# Autodesk Inventor assembly: 装配-载板集合
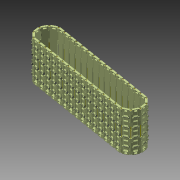
[picture p0: Inventor's stored thumbnail of the model, 180x180]
Saved by Autodesk Inventor 2015 (Build 190159000, 159)
## iProperties
Created: 2017-05-23
Part Number: 装配-载板集合
Document SubType Name: Assembly
Designer: Administrator
Author: Administrator
## Documents named in this file (4)
- C:\Users\Administrator\Desktop\毕设改\装配-载板集合.iam
- C:\Users\Administrator\Desktop\毕设改\装配-载板.iam
- C:\Users\Administrator\Desktop\毕设改\夹具固定销.ipt
- C:\Users\Administrator\Desktop\毕设改\夹具固定销螺丝.ipt
## Components (798 placed, 3 different names)
1. 装配-载板:2 [sub-assembly] — 插入:1, 角度:1, 插入:2, 角度:2, 插入:43, 表面齐平:3
2. 装配-载板:3 [sub-assembly] — 插入:2, 角度:2, 插入:3, 角度:3, 插入:38, 表面齐平:2
3. 装配-载板:4 [sub-assembly] — 插入:3, 插入:4, 角度:3, 角度:4, 插入:36, 插入:37
4. 装配-载板:5 [sub-assembly] — 插入:4, 插入:5, 角度:4, 插入:35, 表面齐平:1
5. 装配-载板:7 [sub-assembly] — 插入:6, 角度:5, 插入:7, 角度:6, 插入:62, 配合:1
6. 装配-载板:8 [sub-assembly] — 插入:6, 角度:5, 插入:9, 插入:60, 插入:61
7. 装配-载板:37 [sub-assembly] — 插入:7, 角度:6, 插入:8, 角度:7, 插入:63, 表面齐平:4
8. 装配-载板:38 [sub-assembly] — 插入:8, 角度:7, 插入:10, 插入:64, 表面齐平:5
9. 装配-载板:1 [sub-assembly] — 插入:1, 角度:1
10. 装配-载板:9 [sub-assembly]
11. 装配-载板:10 [sub-assembly]
12. 装配-载板:11 [sub-assembly]
13. 装配-载板:12 [sub-assembly]
14. 装配-载板:13 [sub-assembly]
15. 装配-载板:14 [sub-assembly]
16. 装配-载板:15 [sub-assembly]
17. 装配-载板:16 [sub-assembly]
18. 装配-载板:17 [sub-assembly]
19. 装配-载板:18 [sub-assembly]
20. 装配-载板:19 [sub-assembly]
21. 装配-载板:20 [sub-assembly]
22. 装配-载板:21 [sub-assembly]
23. 装配-载板:22 [sub-assembly] — 插入:10, 插入:21, 插入:22
24. 装配-载板:6 [sub-assembly] — 插入:5, 插入:11, 插入:12
25. 装配-载板:23 [sub-assembly]
26. 装配-载板:24 [sub-assembly]
27. 装配-载板:25 [sub-assembly]
28. 装配-载板:26 [sub-assembly]
29. 装配-载板:27 [sub-assembly]
30. 装配-载板:28 [sub-assembly]
31. 装配-载板:29 [sub-assembly]
32. 装配-载板:30 [sub-assembly]
33. 装配-载板:31 [sub-assembly]
34. 装配-载板:32 [sub-assembly]
35. 装配-载板:33 [sub-assembly]
36. 装配-载板:34 [sub-assembly]
37. 装配-载板:35 [sub-assembly]
38. 装配-载板:36 [sub-assembly] — 插入:9
39. 夹具固定销:130 — 插入:60, 插入:61
40. 夹具固定销螺丝:502
41. 夹具固定销螺丝:503
42. 夹具固定销螺丝:505
43. 夹具固定销螺丝:504
44. 夹具固定销:133 — 插入:62, 配合:1
45. 夹具固定销螺丝:515
46. 夹具固定销螺丝:514
47. 夹具固定销螺丝:517
48. 夹具固定销螺丝:516
49. 夹具固定销:132 — 插入:64, 表面齐平:5
50. 夹具固定销螺丝:510
51. 夹具固定销螺丝:511
52. 夹具固定销螺丝:513
53. 夹具固定销螺丝:512
54. 夹具固定销:131 — 插入:63, 表面齐平:4
55. 夹具固定销螺丝:506
56. 夹具固定销螺丝:507
57. 夹具固定销螺丝:509
58. 夹具固定销螺丝:508
59. 夹具固定销:128 — 插入:38, 表面齐平:2
60. 夹具固定销螺丝:494
61. 夹具固定销螺丝:495
62. 夹具固定销螺丝:496
63. 夹具固定销螺丝:497
64. 夹具固定销:129 — 插入:43, 表面齐平:3
65. 夹具固定销螺丝:498
66. 夹具固定销螺丝:499
67. 夹具固定销螺丝:501
68. 夹具固定销螺丝:500
69. 夹具固定销:2 — 插入:23, 插入:24, 插入:25, 插入:26, 插入:35, 表面齐平:1
70. 夹具固定销螺丝:2 — 插入:23
71. 夹具固定销螺丝:487 — 插入:26
72. 夹具固定销螺丝:489 — 插入:25
73. 夹具固定销螺丝:488 — 插入:24
74. 夹具固定销:127 — 插入:36, 插入:37
75. 夹具固定销螺丝:490
76. 夹具固定销螺丝:491
77. 夹具固定销螺丝:493
78. 夹具固定销螺丝:492
79. 夹具固定销:134
80. 夹具固定销螺丝:518
81. 夹具固定销螺丝:519
82. 夹具固定销螺丝:520
83. 夹具固定销螺丝:521
84. 夹具固定销:135
85. 夹具固定销螺丝:522
86. 夹具固定销螺丝:523
87. 夹具固定销螺丝:524
88. 夹具固定销螺丝:525
89. 夹具固定销:136
90. 夹具固定销螺丝:526
91. 夹具固定销螺丝:527
92. 夹具固定销螺丝:528
93. 夹具固定销螺丝:529
94. 夹具固定销:137
95. 夹具固定销螺丝:530
96. 夹具固定销螺丝:531
97. 夹具固定销螺丝:532
98. 夹具固定销螺丝:533
99. 夹具固定销:138
100. 夹具固定销螺丝:534
101. 夹具固定销螺丝:535
102. 夹具固定销螺丝:536
103. 夹具固定销螺丝:537
104. 夹具固定销:139
105. 夹具固定销螺丝:538
106. 夹具固定销螺丝:539
107. 夹具固定销螺丝:540
108. 夹具固定销螺丝:541
109. 夹具固定销:140
110. 夹具固定销螺丝:542
111. 夹具固定销螺丝:543
112. 夹具固定销螺丝:544
113. 夹具固定销螺丝:545
114. 夹具固定销:141
115. 夹具固定销螺丝:546
116. 夹具固定销螺丝:547
117. 夹具固定销螺丝:548
118. 夹具固定销螺丝:549
119. 夹具固定销:142
120. 夹具固定销螺丝:550
121. 夹具固定销螺丝:551
122. 夹具固定销螺丝:552
123. 夹具固定销螺丝:553
124. 夹具固定销:143
125. 夹具固定销螺丝:554
126. 夹具固定销螺丝:555
127. 夹具固定销螺丝:556
128. 夹具固定销螺丝:557
129. 夹具固定销:144
130. 夹具固定销螺丝:558
131. 夹具固定销螺丝:559
132. 夹具固定销螺丝:560
133. 夹具固定销螺丝:561
134. 夹具固定销:145
135. 夹具固定销螺丝:562
136. 夹具固定销螺丝:563
137. 夹具固定销螺丝:564
138. 夹具固定销螺丝:565
139. 夹具固定销:146
140. 夹具固定销螺丝:566
141. 夹具固定销螺丝:567
142. 夹具固定销螺丝:568
143. 夹具固定销螺丝:569
144. 夹具固定销:147
145. 夹具固定销螺丝:570
146. 夹具固定销螺丝:571
147. 夹具固定销螺丝:572
148. 夹具固定销螺丝:573
149. 夹具固定销:148
150. 夹具固定销螺丝:574
151. 夹具固定销螺丝:575
152. 夹具固定销螺丝:576
153. 夹具固定销螺丝:577
154. 夹具固定销:149
155. 夹具固定销螺丝:578
156. 夹具固定销螺丝:579
157. 夹具固定销螺丝:580
158. 夹具固定销螺丝:581
159. 夹具固定销:150
160. 夹具固定销螺丝:582
161. 夹具固定销螺丝:583
162. 夹具固定销螺丝:584
163. 夹具固定销螺丝:585
164. 夹具固定销:151
165. 夹具固定销螺丝:586
166. 夹具固定销螺丝:587
167. 夹具固定销螺丝:588
168. 夹具固定销螺丝:589
169. 夹具固定销:152
170. 夹具固定销螺丝:590
171. 夹具固定销螺丝:591
172. 夹具固定销螺丝:592
173. 夹具固定销螺丝:593
174. 夹具固定销:153
175. 夹具固定销螺丝:594
176. 夹具固定销螺丝:595
177. 夹具固定销螺丝:596
178. 夹具固定销螺丝:597
179. 夹具固定销:154
180. 夹具固定销螺丝:598
181. 夹具固定销螺丝:599
182. 夹具固定销螺丝:600
183. 夹具固定销螺丝:601
184. 夹具固定销:155
185. 夹具固定销螺丝:602
186. 夹具固定销螺丝:603
187. 夹具固定销螺丝:604
188. 夹具固定销螺丝:605
189. 夹具固定销:156
190. 夹具固定销螺丝:606
191. 夹具固定销螺丝:607
192. 夹具固定销螺丝:608
193. 夹具固定销螺丝:609
194. 夹具固定销:157
195. 夹具固定销螺丝:610
196. 夹具固定销螺丝:611
197. 夹具固定销螺丝:612
198. 夹具固定销螺丝:613
199. 夹具固定销:5 — 插入:11, 插入:12, 插入:13, 插入:14, 插入:15, 插入:16
200. 夹具固定销螺丝:5 — 插入:13
201. 夹具固定销螺丝:10 — 插入:15
202. 夹具固定销螺丝:11 — 插入:16
203. 夹具固定销螺丝:9 — 插入:14
204. 夹具固定销:9
205. 夹具固定销螺丝:12
206. 夹具固定销螺丝:13
207. 夹具固定销螺丝:14
208. 夹具固定销螺丝:15
209. 夹具固定销:10
210. 夹具固定销螺丝:16
211. 夹具固定销螺丝:17
212. 夹具固定销螺丝:18
213. 夹具固定销螺丝:19
214. 夹具固定销:11
215. 夹具固定销螺丝:20
216. 夹具固定销螺丝:21
217. 夹具固定销螺丝:22
218. 夹具固定销螺丝:23
219. 夹具固定销:12
220. 夹具固定销螺丝:24
221. 夹具固定销螺丝:25
222. 夹具固定销螺丝:26
223. 夹具固定销螺丝:27
224. 夹具固定销:13
225. 夹具固定销螺丝:28
226. 夹具固定销螺丝:29
227. 夹具固定销螺丝:30
228. 夹具固定销螺丝:31
229. 夹具固定销:14
230. 夹具固定销螺丝:32
231. 夹具固定销螺丝:33
232. 夹具固定销螺丝:34
233. 夹具固定销螺丝:35
234. 夹具固定销:15
235. 夹具固定销螺丝:36
236. 夹具固定销螺丝:37
237. 夹具固定销螺丝:38
238. 夹具固定销螺丝:39
239. 夹具固定销:16
240. 夹具固定销螺丝:40
241. 夹具固定销螺丝:41
242. 夹具固定销螺丝:42
243. 夹具固定销螺丝:43
244. 夹具固定销:17
245. 夹具固定销螺丝:44
246. 夹具固定销螺丝:45
247. 夹具固定销螺丝:46
248. 夹具固定销螺丝:47
249. 夹具固定销:18
250. 夹具固定销螺丝:48
251. 夹具固定销螺丝:49
252. 夹具固定销螺丝:50
253. 夹具固定销螺丝:51
254. 夹具固定销:19
255. 夹具固定销螺丝:52
256. 夹具固定销螺丝:53
257. 夹具固定销螺丝:54
258. 夹具固定销螺丝:55
259. 夹具固定销:20
260. 夹具固定销螺丝:56
261. 夹具固定销螺丝:57
262. 夹具固定销螺丝:58
263. 夹具固定销螺丝:59
264. 夹具固定销:21
265. 夹具固定销螺丝:60
266. 夹具固定销螺丝:61
267. 夹具固定销螺丝:62
268. 夹具固定销螺丝:63
269. 夹具固定销:22
270. 夹具固定销螺丝:64
271. 夹具固定销螺丝:65
272. 夹具固定销螺丝:66
273. 夹具固定销螺丝:67
274. 夹具固定销:23
275. 夹具固定销螺丝:68
276. 夹具固定销螺丝:69
277. 夹具固定销螺丝:70
278. 夹具固定销螺丝:71
279. 夹具固定销:24
280. 夹具固定销螺丝:72
281. 夹具固定销螺丝:73
282. 夹具固定销螺丝:74
283. 夹具固定销螺丝:75
284. 夹具固定销:25
285. 夹具固定销螺丝:76
286. 夹具固定销螺丝:77
287. 夹具固定销螺丝:78
288. 夹具固定销螺丝:79
289. 夹具固定销:26
290. 夹具固定销螺丝:80
291. 夹具固定销螺丝:81
292. 夹具固定销螺丝:82
293. 夹具固定销螺丝:83
294. 夹具固定销:27
295. 夹具固定销螺丝:84
296. 夹具固定销螺丝:85
297. 夹具固定销螺丝:86
298. 夹具固定销螺丝:87
299. 夹具固定销:28
300. 夹具固定销螺丝:88
301. 夹具固定销螺丝:89
302. 夹具固定销螺丝:90
303. 夹具固定销螺丝:91
304. 夹具固定销:29
305. 夹具固定销螺丝:92
306. 夹具固定销螺丝:93
307. 夹具固定销螺丝:94
308. 夹具固定销螺丝:95
309. 夹具固定销:30
310. 夹具固定销螺丝:96
311. 夹具固定销螺丝:97
312. 夹具固定销螺丝:98
313. 夹具固定销螺丝:99
314. 夹具固定销:31
315. 夹具固定销螺丝:100
316. 夹具固定销螺丝:101
317. 夹具固定销螺丝:102
318. 夹具固定销螺丝:103
319. 夹具固定销:32
320. 夹具固定销螺丝:104
321. 夹具固定销螺丝:105
322. 夹具固定销螺丝:106
323. 夹具固定销螺丝:107
324. 夹具固定销:33
325. 夹具固定销螺丝:108
326. 夹具固定销螺丝:109
327. 夹具固定销螺丝:110
328. 夹具固定销螺丝:111
329. 夹具固定销:34
330. 夹具固定销螺丝:112
331. 夹具固定销螺丝:113
332. 夹具固定销螺丝:114
333. 夹具固定销螺丝:115
334. 夹具固定销:35
335. 夹具固定销螺丝:116
336. 夹具固定销螺丝:117
337. 夹具固定销螺丝:118
338. 夹具固定销螺丝:119
339. 夹具固定销:36
340. 夹具固定销螺丝:120
341. 夹具固定销螺丝:121
342. 夹具固定销螺丝:122
343. 夹具固定销螺丝:123
344. 夹具固定销:37
345. 夹具固定销螺丝:124
346. 夹具固定销螺丝:125
347. 夹具固定销螺丝:126
348. 夹具固定销螺丝:127
349. 夹具固定销:38
350. 夹具固定销螺丝:128
351. 夹具固定销螺丝:129
352. 夹具固定销螺丝:130
353. 夹具固定销螺丝:131
354. 夹具固定销:39
355. 夹具固定销螺丝:132
356. 夹具固定销螺丝:133
357. 夹具固定销螺丝:134
358. 夹具固定销螺丝:135
359. 夹具固定销:40
360. 夹具固定销螺丝:136
361. 夹具固定销螺丝:137
362. 夹具固定销螺丝:138
363. 夹具固定销螺丝:139
364. 夹具固定销:41
365. 夹具固定销螺丝:140
366. 夹具固定销螺丝:141
367. 夹具固定销螺丝:142
368. 夹具固定销螺丝:143
369. 夹具固定销:42
370. 夹具固定销螺丝:144
371. 夹具固定销螺丝:145
372. 夹具固定销螺丝:146
373. 夹具固定销螺丝:147
374. 夹具固定销:43
375. 夹具固定销螺丝:148
376. 夹具固定销螺丝:149
377. 夹具固定销螺丝:150
378. 夹具固定销螺丝:151
379. 夹具固定销:44
380. 夹具固定销螺丝:152
381. 夹具固定销螺丝:153
382. 夹具固定销螺丝:154
383. 夹具固定销螺丝:155
384. 夹具固定销:45
385. 夹具固定销螺丝:156
386. 夹具固定销螺丝:157
387. 夹具固定销螺丝:158
388. 夹具固定销螺丝:159
389. 夹具固定销:46
390. 夹具固定销螺丝:160
391. 夹具固定销螺丝:161
392. 夹具固定销螺丝:162
393. 夹具固定销螺丝:163
394. 夹具固定销:47
395. 夹具固定销螺丝:164
396. 夹具固定销螺丝:165
397. 夹具固定销螺丝:166
398. 夹具固定销螺丝:167
399. 夹具固定销:48
400. 夹具固定销螺丝:168
401. 夹具固定销螺丝:169
402. 夹具固定销螺丝:170
403. 夹具固定销螺丝:171
404. 夹具固定销:49
405. 夹具固定销螺丝:172
406. 夹具固定销螺丝:173
407. 夹具固定销螺丝:174
408. 夹具固定销螺丝:175
409. 夹具固定销:50
410. 夹具固定销螺丝:176
411. 夹具固定销螺丝:177
412. 夹具固定销螺丝:178
413. 夹具固定销螺丝:179
414. 夹具固定销:51
415. 夹具固定销螺丝:180
416. 夹具固定销螺丝:181
417. 夹具固定销螺丝:182
418. 夹具固定销螺丝:183
419. 夹具固定销:52
420. 夹具固定销螺丝:184
421. 夹具固定销螺丝:185
422. 夹具固定销螺丝:186
423. 夹具固定销螺丝:187
424. 夹具固定销:53
425. 夹具固定销螺丝:188
426. 夹具固定销螺丝:189
427. 夹具固定销螺丝:190
428. 夹具固定销螺丝:191
429. 夹具固定销:54
430. 夹具固定销螺丝:192
431. 夹具固定销螺丝:193
432. 夹具固定销螺丝:194
433. 夹具固定销螺丝:195
434. 夹具固定销:55
435. 夹具固定销螺丝:196
436. 夹具固定销螺丝:197
437. 夹具固定销螺丝:198
438. 夹具固定销螺丝:199
439. 夹具固定销:56
440. 夹具固定销螺丝:200
441. 夹具固定销螺丝:201
442. 夹具固定销螺丝:202
443. 夹具固定销螺丝:203
444. 夹具固定销:57
445. 夹具固定销螺丝:204
446. 夹具固定销螺丝:205
447. 夹具固定销螺丝:206
448. 夹具固定销螺丝:207
449. 夹具固定销:58
450. 夹具固定销螺丝:208
451. 夹具固定销螺丝:209
452. 夹具固定销螺丝:210
453. 夹具固定销螺丝:211
454. 夹具固定销:59
455. 夹具固定销螺丝:212
456. 夹具固定销螺丝:213
457. 夹具固定销螺丝:214
458. 夹具固定销螺丝:215
459. 夹具固定销:60
460. 夹具固定销螺丝:216
461. 夹具固定销螺丝:217
462. 夹具固定销螺丝:218
463. 夹具固定销螺丝:219
464. 夹具固定销:61
465. 夹具固定销螺丝:220
466. 夹具固定销螺丝:221
467. 夹具固定销螺丝:222
468. 夹具固定销螺丝:223
469. 夹具固定销:62
470. 夹具固定销螺丝:224
471. 夹具固定销螺丝:225
472. 夹具固定销螺丝:226
473. 夹具固定销螺丝:227
474. 夹具固定销:63
475. 夹具固定销螺丝:228
476. 夹具固定销螺丝:229
477. 夹具固定销螺丝:230
478. 夹具固定销螺丝:231
479. 夹具固定销:64
480. 夹具固定销螺丝:232
481. 夹具固定销螺丝:233
482. 夹具固定销螺丝:234
483. 夹具固定销螺丝:235
484. 夹具固定销:65
485. 夹具固定销螺丝:236
486. 夹具固定销螺丝:237
487. 夹具固定销螺丝:238
488. 夹具固定销螺丝:239
489. 夹具固定销:66
490. 夹具固定销螺丝:240
491. 夹具固定销螺丝:241
492. 夹具固定销螺丝:242
493. 夹具固定销螺丝:243
494. 夹具固定销:67
495. 夹具固定销螺丝:244
496. 夹具固定销螺丝:245
497. 夹具固定销螺丝:246
498. 夹具固定销螺丝:247
499. 夹具固定销:1 — 插入:17, 插入:18, 插入:19, 插入:20, 插入:21, 插入:22
500. 夹具固定销螺丝:249 — 插入:18
501. 夹具固定销螺丝:1 — 插入:17
502. 夹具固定销螺丝:250 — 插入:20
503. 夹具固定销螺丝:248 — 插入:19
504. 夹具固定销:68
505. 夹具固定销螺丝:251
506. 夹具固定销螺丝:252
507. 夹具固定销螺丝:253
508. 夹具固定销螺丝:254
509. 夹具固定销:69
510. 夹具固定销螺丝:255
511. 夹具固定销螺丝:256
512. 夹具固定销螺丝:257
513. 夹具固定销螺丝:258
514. 夹具固定销:70
515. 夹具固定销螺丝:259
516. 夹具固定销螺丝:260
517. 夹具固定销螺丝:261
518. 夹具固定销螺丝:262
519. 夹具固定销:71
520. 夹具固定销螺丝:263
521. 夹具固定销螺丝:264
522. 夹具固定销螺丝:265
523. 夹具固定销螺丝:266
524. 夹具固定销:72
525. 夹具固定销螺丝:267
526. 夹具固定销螺丝:268
527. 夹具固定销螺丝:269
528. 夹具固定销螺丝:270
529. 夹具固定销:73
530. 夹具固定销螺丝:271
531. 夹具固定销螺丝:272
532. 夹具固定销螺丝:273
533. 夹具固定销螺丝:274
534. 夹具固定销:74
535. 夹具固定销螺丝:275
536. 夹具固定销螺丝:276
537. 夹具固定销螺丝:277
538. 夹具固定销螺丝:278
539. 夹具固定销:75
540. 夹具固定销螺丝:279
541. 夹具固定销螺丝:280
542. 夹具固定销螺丝:281
543. 夹具固定销螺丝:282
544. 夹具固定销:76
545. 夹具固定销螺丝:283
546. 夹具固定销螺丝:284
547. 夹具固定销螺丝:285
548. 夹具固定销螺丝:286
549. 夹具固定销:77
550. 夹具固定销螺丝:287
551. 夹具固定销螺丝:288
552. 夹具固定销螺丝:289
553. 夹具固定销螺丝:290
554. 夹具固定销:78
555. 夹具固定销螺丝:291
556. 夹具固定销螺丝:292
557. 夹具固定销螺丝:293
558. 夹具固定销螺丝:294
559. 夹具固定销:79
560. 夹具固定销螺丝:295
561. 夹具固定销螺丝:296
562. 夹具固定销螺丝:297
563. 夹具固定销螺丝:298
564. 夹具固定销:80
565. 夹具固定销螺丝:299
566. 夹具固定销螺丝:300
567. 夹具固定销螺丝:301
568. 夹具固定销螺丝:302
569. 夹具固定销:81
570. 夹具固定销螺丝:303
571. 夹具固定销螺丝:304
572. 夹具固定销螺丝:305
573. 夹具固定销螺丝:306
574. 夹具固定销:82
575. 夹具固定销螺丝:307
576. 夹具固定销螺丝:308
577. 夹具固定销螺丝:309
578. 夹具固定销螺丝:310
579. 夹具固定销:83
580. 夹具固定销螺丝:311
581. 夹具固定销螺丝:312
582. 夹具固定销螺丝:313
583. 夹具固定销螺丝:314
584. 夹具固定销:84
585. 夹具固定销螺丝:315
586. 夹具固定销螺丝:316
587. 夹具固定销螺丝:317
588. 夹具固定销螺丝:318
589. 夹具固定销:85
590. 夹具固定销螺丝:319
591. 夹具固定销螺丝:320
592. 夹具固定销螺丝:321
593. 夹具固定销螺丝:322
594. 夹具固定销:86
595. 夹具固定销螺丝:323
596. 夹具固定销螺丝:324
597. 夹具固定销螺丝:325
598. 夹具固定销螺丝:326
599. 夹具固定销:87
600. 夹具固定销螺丝:327
601. 夹具固定销螺丝:328
602. 夹具固定销螺丝:329
603. 夹具固定销螺丝:330
604. 夹具固定销:88
605. 夹具固定销螺丝:331
606. 夹具固定销螺丝:332
607. 夹具固定销螺丝:333
608. 夹具固定销螺丝:334
609. 夹具固定销:89
610. 夹具固定销螺丝:335
611. 夹具固定销螺丝:336
612. 夹具固定销螺丝:337
613. 夹具固定销螺丝:338
614. 夹具固定销:90
615. 夹具固定销螺丝:339
616. 夹具固定销螺丝:340
617. 夹具固定销螺丝:341
618. 夹具固定销螺丝:342
619. 夹具固定销:91
620. 夹具固定销螺丝:343
621. 夹具固定销螺丝:344
622. 夹具固定销螺丝:345
623. 夹具固定销螺丝:346
624. 夹具固定销:92
625. 夹具固定销螺丝:347
626. 夹具固定销螺丝:348
627. 夹具固定销螺丝:349
628. 夹具固定销螺丝:350
629. 夹具固定销:93
630. 夹具固定销螺丝:351
631. 夹具固定销螺丝:352
632. 夹具固定销螺丝:353
633. 夹具固定销螺丝:354
634. 夹具固定销:94
635. 夹具固定销螺丝:355
636. 夹具固定销螺丝:356
637. 夹具固定销螺丝:357
638. 夹具固定销螺丝:358
639. 夹具固定销:95
640. 夹具固定销螺丝:359
641. 夹具固定销螺丝:360
642. 夹具固定销螺丝:361
643. 夹具固定销螺丝:362
644. 夹具固定销:96
645. 夹具固定销螺丝:363
646. 夹具固定销螺丝:364
647. 夹具固定销螺丝:365
648. 夹具固定销螺丝:366
649. 夹具固定销:97
650. 夹具固定销螺丝:367
651. 夹具固定销螺丝:368
652. 夹具固定销螺丝:369
653. 夹具固定销螺丝:370
654. 夹具固定销:98
655. 夹具固定销螺丝:371
656. 夹具固定销螺丝:372
657. 夹具固定销螺丝:373
658. 夹具固定销螺丝:374
659. 夹具固定销:99
660. 夹具固定销螺丝:375
661. 夹具固定销螺丝:376
662. 夹具固定销螺丝:377
663. 夹具固定销螺丝:378
664. 夹具固定销:100
665. 夹具固定销螺丝:379
666. 夹具固定销螺丝:380
667. 夹具固定销螺丝:381
668. 夹具固定销螺丝:382
669. 夹具固定销:101
670. 夹具固定销螺丝:383
671. 夹具固定销螺丝:384
672. 夹具固定销螺丝:385
673. 夹具固定销螺丝:386
674. 夹具固定销:102
675. 夹具固定销螺丝:387
676. 夹具固定销螺丝:388
677. 夹具固定销螺丝:389
678. 夹具固定销螺丝:390
679. 夹具固定销:103
680. 夹具固定销螺丝:391
681. 夹具固定销螺丝:392
682. 夹具固定销螺丝:393
683. 夹具固定销螺丝:394
684. 夹具固定销:104
685. 夹具固定销螺丝:395
686. 夹具固定销螺丝:396
687. 夹具固定销螺丝:397
688. 夹具固定销螺丝:398
689. 夹具固定销:105
690. 夹具固定销螺丝:399
691. 夹具固定销螺丝:400
692. 夹具固定销螺丝:401
693. 夹具固定销螺丝:402
694. 夹具固定销:106
695. 夹具固定销螺丝:403
696. 夹具固定销螺丝:404
697. 夹具固定销螺丝:405
698. 夹具固定销螺丝:406
699. 夹具固定销:107
700. 夹具固定销螺丝:407
701. 夹具固定销螺丝:408
702. 夹具固定销螺丝:409
703. 夹具固定销螺丝:410
704. 夹具固定销:108
705. 夹具固定销螺丝:411
706. 夹具固定销螺丝:412
707. 夹具固定销螺丝:413
708. 夹具固定销螺丝:414
709. 夹具固定销:109
710. 夹具固定销螺丝:415
711. 夹具固定销螺丝:416
712. 夹具固定销螺丝:417
713. 夹具固定销螺丝:418
714. 夹具固定销:110
715. 夹具固定销螺丝:419
716. 夹具固定销螺丝:420
717. 夹具固定销螺丝:421
718. 夹具固定销螺丝:422
719. 夹具固定销:111
720. 夹具固定销螺丝:423
721. 夹具固定销螺丝:424
722. 夹具固定销螺丝:425
723. 夹具固定销螺丝:426
724. 夹具固定销:112
725. 夹具固定销螺丝:427
726. 夹具固定销螺丝:428
727. 夹具固定销螺丝:429
728. 夹具固定销螺丝:430
729. 夹具固定销:113
730. 夹具固定销螺丝:431
731. 夹具固定销螺丝:432
732. 夹具固定销螺丝:433
733. 夹具固定销螺丝:434
734. 夹具固定销:114
735. 夹具固定销螺丝:435
736. 夹具固定销螺丝:436
737. 夹具固定销螺丝:437
738. 夹具固定销螺丝:438
739. 夹具固定销:115
740. 夹具固定销螺丝:439
741. 夹具固定销螺丝:440
742. 夹具固定销螺丝:441
743. 夹具固定销螺丝:442
744. 夹具固定销:116
745. 夹具固定销螺丝:443
746. 夹具固定销螺丝:444
747. 夹具固定销螺丝:445
748. 夹具固定销螺丝:446
749. 夹具固定销:117
750. 夹具固定销螺丝:447
751. 夹具固定销螺丝:448
752. 夹具固定销螺丝:449
753. 夹具固定销螺丝:450
754. 夹具固定销:118
755. 夹具固定销螺丝:451
756. 夹具固定销螺丝:452
757. 夹具固定销螺丝:453
758. 夹具固定销螺丝:454
759. 夹具固定销:119
760. 夹具固定销螺丝:455
761. 夹具固定销螺丝:456
762. 夹具固定销螺丝:457
763. 夹具固定销螺丝:458
764. 夹具固定销:120
765. 夹具固定销螺丝:459
766. 夹具固定销螺丝:460
767. 夹具固定销螺丝:461
768. 夹具固定销螺丝:462
769. 夹具固定销:121
770. 夹具固定销螺丝:463
771. 夹具固定销螺丝:464
772. 夹具固定销螺丝:465
773. 夹具固定销螺丝:466
774. 夹具固定销:122
775. 夹具固定销螺丝:467
776. 夹具固定销螺丝:468
777. 夹具固定销螺丝:469
778. 夹具固定销螺丝:470
779. 夹具固定销:123
780. 夹具固定销螺丝:471
781. 夹具固定销螺丝:472
782. 夹具固定销螺丝:473
783. 夹具固定销螺丝:474
784. 夹具固定销:124
785. 夹具固定销螺丝:475
786. 夹具固定销螺丝:476
787. 夹具固定销螺丝:477
788. 夹具固定销螺丝:478
789. 夹具固定销:125
790. 夹具固定销螺丝:479
791. 夹具固定销螺丝:480
792. 夹具固定销螺丝:481
793. 夹具固定销螺丝:482
794. 夹具固定销:126
795. 夹具固定销螺丝:483
796. 夹具固定销螺丝:484
797. 夹具固定销螺丝:485
798. 夹具固定销螺丝:486
## Component patterns: (15 elements, first: 装配-载板:1), (15 elements, first: 装配-载板:6), (15 elements), (15 elements), (4 elements, first: 夹具固定销:130 + 夹具固定销螺丝:502 + 夹具固定销螺丝:503 + 夹具固定销螺丝:505 + 夹具固定销螺丝:504 + 夹具固定销:133 + 夹具固定销螺丝:515 + 夹具固定销螺丝:514 + 夹具固定销螺丝:517 + 夹具固定销螺丝:516 + 夹具固定销:132 + 夹具固定销螺丝:510 + 夹具固定销螺丝:511 + 夹具固定销螺丝:513 + 夹具固定销螺丝:512 + 夹具固定销:131 + 夹具固定销螺丝:506 + 夹具固定销螺丝:507 + 夹具固定销螺丝:509 + 夹具固定销螺丝:508 + 夹具固定销:128 + 夹具固定销螺丝:494 + 夹具固定销螺丝:495 + 夹具固定销螺丝:496 + 夹具固定销螺丝:497 + 夹具固定销:129 + 夹具固定销螺丝:498 + 夹具固定销螺丝:499 + 夹具固定销螺丝:501 + 夹具固定销螺丝:500 + 夹具固定销:2 + 夹具固定销螺丝:2 + 夹具固定销螺丝:487 + 夹具固定销螺丝:489 + 夹具固定销螺丝:488 + 夹具固定销:127 + 夹具固定销螺丝:490 + 夹具固定销螺丝:491 + 夹具固定销螺丝:493 + 夹具固定销螺丝:492), (4 elements, first: 夹具固定销:5 + 夹具固定销螺丝:5 + 夹具固定销螺丝:10 + 夹具固定销螺丝:11 + 夹具固定销螺丝:9), 零部件阵列 3:2 (4 elements), 零部件阵列 3:3 (4 elements), 零部件阵列 3:4 (4 elements), 零部件阵列 3:5 (4 elements), 零部件阵列 3:6 (4 elements), 零部件阵列 3:7 (4 elements), 零部件阵列 3:8 (4 elements), 零部件阵列 3:9 (4 elements), 零部件阵列 3:10 (4 elements), 零部件阵列 3:11 (4 elements), 零部件阵列 3:12 (4 elements), 零部件阵列 3:13 (4 elements), 零部件阵列 3:14 (4 elements), 零部件阵列 3:15 (4 elements), (4 elements, first: 夹具固定销:1 + 夹具固定销螺丝:249 + 夹具固定销螺丝:1 + 夹具固定销螺丝:250 + 夹具固定销螺丝:248), 零部件阵列 5:2 (4 elements), 零部件阵列 5:3 (4 elements), 零部件阵列 5:4 (4 elements), 零部件阵列 5:5 (4 elements), 零部件阵列 5:6 (4 elements), 零部件阵列 5:7 (4 elements), 零部件阵列 5:8 (4 elements), 零部件阵列 5:9 (4 elements), 零部件阵列 5:10 (4 elements), 零部件阵列 5:11 (4 elements), 零部件阵列 5:12 (4 elements), 零部件阵列 5:13 (4 elements), 零部件阵列 5:14 (4 elements), 零部件阵列 5:15 (4 elements)
## Relationships (77: Insert 64, Angle 7, Flush 5, Mate 1)
- 插入:1 [Insert]: 装配-载板:2 ↔ 装配-载板:1
- 角度:1 [Angle] (36 deg): 装配-载板:2 ↔ 装配-载板:1
- 插入:2 [Insert]: 装配-载板:2 ↔ 装配-载板:3
- 角度:2 [Angle] (36 deg): 装配-载板:2 ↔ 装配-载板:3
- 插入:3 [Insert]: 装配-载板:3 ↔ 装配-载板:4
- 插入:4 [Insert]: 装配-载板:4 ↔ 装配-载板:5
- 插入:5 [Insert]: 装配-载板:5 ↔ 装配-载板:6
- 角度:3 [Angle] (36 deg): 装配-载板:3 ↔ 装配-载板:4
- 角度:4 [Angle] (36 deg): 装配-载板:4 ↔ 装配-载板:5
- 插入:6 [Insert]: 装配-载板:7 ↔ 装配-载板:8
- 角度:5 [Angle] (36 deg): 装配-载板:7 ↔ 装配-载板:8
- 插入:7 [Insert]: 装配-载板:7 ↔ 装配-载板:37
- 角度:6 [Angle] (36 deg): 装配-载板:7 ↔ 装配-载板:37
- 插入:8 [Insert]: 装配-载板:37 ↔ 装配-载板:38
- 角度:7 [Angle] (36 deg): 装配-载板:37 ↔ 装配-载板:38
- 插入:9 [Insert]: 装配-载板:8 ↔ 装配-载板:36
- 插入:10 [Insert]: 装配-载板:38 ↔ 装配-载板:22
- 插入:11 [Insert]: 装配-载板:6 ↔ 夹具固定销:5
- 插入:12 [Insert]: 装配-载板:6 ↔ 夹具固定销:5
- 插入:13 [Insert]: 夹具固定销:5 ↔ 夹具固定销螺丝:5
- 插入:14 [Insert]: 夹具固定销:5 ↔ 夹具固定销螺丝:9
- 插入:15 [Insert]: 夹具固定销:5 ↔ 夹具固定销螺丝:10
- 插入:16 [Insert]: 夹具固定销:5 ↔ 夹具固定销螺丝:11
- 插入:17 [Insert]: 夹具固定销:1 ↔ 夹具固定销螺丝:1
- 插入:18 [Insert]: 夹具固定销:1 ↔ 夹具固定销螺丝:249
- 插入:19 [Insert]: 夹具固定销:1 ↔ 夹具固定销螺丝:248
- 插入:20 [Insert]: 夹具固定销:1 ↔ 夹具固定销螺丝:250
- 插入:21 [Insert]: 装配-载板:22 ↔ 夹具固定销:1
- 插入:22 [Insert]: 装配-载板:22 ↔ 夹具固定销:1
- 插入:23 [Insert]: 夹具固定销:2 ↔ 夹具固定销螺丝:2
- 插入:24 [Insert]: 夹具固定销:2 ↔ 夹具固定销螺丝:488
- 插入:25 [Insert]: 夹具固定销:2 ↔ 夹具固定销螺丝:489
- 插入:26 [Insert]: 夹具固定销:2 ↔ 夹具固定销螺丝:487
- [Insert]: 夹具固定销:127 ↔ 夹具固定销螺丝:490
- [Insert]: 夹具固定销:127 ↔ 夹具固定销螺丝:492
- [Insert]: 夹具固定销:127 ↔ 夹具固定销螺丝:493
- [Insert]: 夹具固定销:127 ↔ 夹具固定销螺丝:491
- [Insert]: 夹具固定销:128 ↔ 夹具固定销螺丝:494
- [Insert]: 夹具固定销:128 ↔ 夹具固定销螺丝:496
- [Insert]: 夹具固定销:128 ↔ 夹具固定销螺丝:497
- [Insert]: 夹具固定销:128 ↔ 夹具固定销螺丝:495
- 插入:35 [Insert]: 装配-载板:5 ↔ 夹具固定销:2
- 表面齐平:1 [Flush]: 装配-载板:5 ↔ 夹具固定销:2
- 插入:36 [Insert]: 装配-载板:4 ↔ 夹具固定销:127
- 插入:37 [Insert]: 装配-载板:4 ↔ 夹具固定销:127
- 插入:38 [Insert]: 装配-载板:3 ↔ 夹具固定销:128
- 表面齐平:2 [Flush]: 装配-载板:3 ↔ 夹具固定销:128
- [Insert]: 夹具固定销:129 ↔ 夹具固定销螺丝:498
- [Insert]: 夹具固定销:129 ↔ 夹具固定销螺丝:500
- [Insert]: 夹具固定销:129 ↔ 夹具固定销螺丝:501
- [Insert]: 夹具固定销:129 ↔ 夹具固定销螺丝:499
- 插入:43 [Insert]: 装配-载板:2 ↔ 夹具固定销:129
- 表面齐平:3 [Flush]: 装配-载板:2 ↔ 夹具固定销:129
- [Insert]: 夹具固定销:130 ↔ 夹具固定销螺丝:502
- [Insert]: 夹具固定销:130 ↔ 夹具固定销螺丝:504
- [Insert]: 夹具固定销:130 ↔ 夹具固定销螺丝:505
- [Insert]: 夹具固定销:130 ↔ 夹具固定销螺丝:503
- [Insert]: 夹具固定销:131 ↔ 夹具固定销螺丝:506
- [Insert]: 夹具固定销:131 ↔ 夹具固定销螺丝:508
- [Insert]: 夹具固定销:131 ↔ 夹具固定销螺丝:509
- [Insert]: 夹具固定销:131 ↔ 夹具固定销螺丝:507
- [Insert]: 夹具固定销:132 ↔ 夹具固定销螺丝:510
- [Insert]: 夹具固定销:132 ↔ 夹具固定销螺丝:512
- [Insert]: 夹具固定销:132 ↔ 夹具固定销螺丝:513
- [Insert]: 夹具固定销:132 ↔ 夹具固定销螺丝:511
- [Insert]: 夹具固定销:133 ↔ 夹具固定销螺丝:514
- [Insert]: 夹具固定销:133 ↔ 夹具固定销螺丝:516
- [Insert]: 夹具固定销:133 ↔ 夹具固定销螺丝:517
- [Insert]: 夹具固定销:133 ↔ 夹具固定销螺丝:515
- 插入:60 [Insert]: 装配-载板:8 ↔ 夹具固定销:130
- 插入:61 [Insert]: 装配-载板:8 ↔ 夹具固定销:130
- 插入:62 [Insert]: 装配-载板:7 ↔ 夹具固定销:133
- 配合:1 [Mate]: 装配-载板:7 ↔ 夹具固定销:133
- 插入:63 [Insert]: 装配-载板:37 ↔ 夹具固定销:131
- 表面齐平:4 [Flush]: 装配-载板:37 ↔ 夹具固定销:131
- 插入:64 [Insert]: 装配-载板:38 ↔ 夹具固定销:132
- 表面齐平:5 [Flush]: 装配-载板:38 ↔ 夹具固定销:132
## Named parameters: d57_d53 = 0 mm, d58_d54 = 0 mm, d59_d55 = 0 mm, d60_d56 = 0 mm, d61_d53 = 0 mm, d62_d54 = 0 mm, d63_d55 = 0 mm, d64_d56 = 0 mm, d71_d53 = 0 mm, d72_d54 = 0 mm, d73_d55 = 0 mm, d74_d56 = 0 mm, d77_d53 = 0 mm, d78_d54 = 0 mm, d79_d55 = 0 mm, d80_d56 = 0 mm, d81_d53 = 0 mm, d82_d54 = 0 mm, d83_d55 = 0 mm, d84_d56 = 0 mm, d85_d53 = 0 mm, d86_d54 = 0 mm, d87_d55 = 0 mm, d88_d56 = 0 mm, d89_d53 = 0 mm, d90_d54 = 0 mm, d91_d55 = 0 mm, d92_d56 = 0 mm
